# Autodesk Inventor assembly: s-assy-shooter_unit
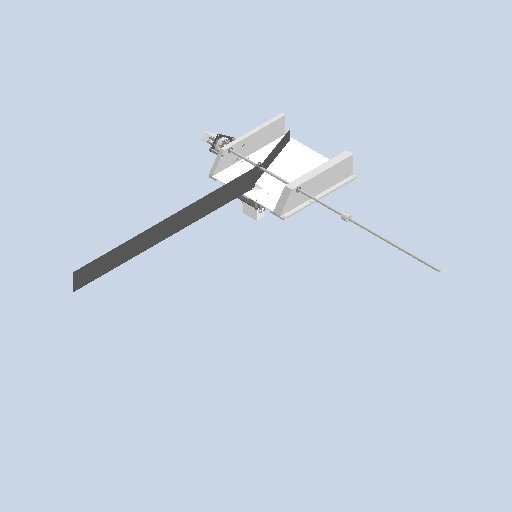
[picture p0: Inventor's stored thumbnail of the model, 512x512]
Saved by Autodesk Inventor 2022 (Build 260153000, 153)
## iProperties
Created: 2021-08-20
Part Number: s-assy-shooter_unit
Document SubType Name: Assembly
Designer: yuta0
Author: yuta0
## Documents named in this file (13)
- C:\Users\yuto6\Box\Public_Share\キャチロボバトルコンテスト2021\CAD\catchrobo_hardware\assy-shooter\s-assy-shooter_unit.iam
- C:\Users\yuto6\Box\Public_Share\キャチロボバトルコンテスト2021\CAD\catchrobo_hardware\assy-shooter\s_carbon_plate1.ipt
- C:\Users\yuto6\Box\Public_Share\キャチロボバトルコンテスト2021\CAD\catchrobo_hardware\assy-shooter\s_base2.ipt
- C:\Users\yuto6\Box\Public_Share\キャチロボバトルコンテスト2021\CAD\catchrobo_hardware\assy-shooter\s_base4.ipt
- C:\Users\yuto6\Box\Public_Share\キャチロボバトルコンテスト2021\CAD\catchrobo_hardware\assy-shooter\s-assy-guide_actuator.iam
- C:\Users\yuto6\Box\Public_Share\キャチロボバトルコンテスト2021\CAD\catchrobo_hardware\assy-shooter\MF126ZZ.ipt
- C:\Users\yuto6\Box\Public_Share\キャチロボバトルコンテスト2021\CAD\catchrobo_hardware\assy-shooter\CPRC16-6-6.iam
- C:\Users\yuto6\Box\Public_Share\キャチロボバトルコンテスト2021\CAD\catchrobo_hardware\assy-shooter\SCSTR6-8.iam
- C:\Users\yuto6\Box\Public_Share\キャチロボバトルコンテスト2021\CAD\catchrobo_hardware\assy-robot\CB4-10.ipt
- C:\Users\yuto6\Box\Public_Share\キャチロボバトルコンテスト2021\CAD\catchrobo_hardware\assy-shooter\s_carbon_plate5.ipt
- C:\Users\yuto6\Box\Public_Share\キャチロボバトルコンテスト2021\CAD\catchrobo_hardware\assy-shooter\s-assy-sorter.iam
- C:\Users\yuto6\Box\Public_Share\キャチロボバトルコンテスト2021\CAD\catchrobo_hardware\assy-shooter\PSFG6-350.ipt
- C:\Users\yuto6\Box\Public_Share\キャチロボバトルコンテスト2021\CAD\catchrobo_hardware\assy-shooter\PSFG6-270.ipt
## Components (17 placed, 12 different names)
1. s_base4:1 — メイト:20, メイト:21, フラッシュ:6, メイト:51, メイト:53, メイト:54, メイト:55, メイト:56, メイト:69, メイト:70, メイト:71, メイト:72, メイト:73, メイト:74, メイト:75, メイト:76, メイト:79
2. s-assy-guide_actuator:1 [sub-assembly] — メイト:51, メイト:69, メイト:70, フラッシュ:7
3. MF126ZZ:1 — メイト:53, メイト:54
4. MF126ZZ:2 — メイト:55, メイト:56
5. MF126ZZ:3 — メイト:58, メイト:59, メイト:83
6. MF126ZZ:4 — メイト:60, メイト:61, メイト:84
7. CPRC16-6-6:1 [sub-assembly] — メイト:65, メイト:84
8. CB4-10:1 — メイト:71, メイト:72
9. CB4-10:2 — メイト:73, メイト:74
10. CB4-10:3 — メイト:75, メイト:76
11. s_carbon_plate5:1 — メイト:78, メイト:79, 角度:1
12. SCSTR6-8:1 [sub-assembly] — メイト:78
13. s_base2:1 — メイト:13, メイト:14, フラッシュ:5, メイト:58, メイト:59, メイト:60, メイト:61, メイト:65
14. s_carbon_plate1:1 — メイト:13, メイト:14, メイト:20, メイト:21, フラッシュ:5, フラッシュ:6, メイト:80, メイト:81, メイト:82, 角度:1
15. s-assy-sorter:1 [sub-assembly] — メイト:80, メイト:81, メイト:82
16. PSFG6-350:1 — メイト:83, フラッシュ:7, メイト:85, メイト:86
17. PSFG6-270:1 — メイト:85, メイト:86
## Relationships (35: Mate 31, Flush 3, Angle 1)
- メイト:13 [Mate]: s_base2:1 ↔ s_carbon_plate1:1
- メイト:14 [Mate]: s_base2:1 ↔ s_carbon_plate1:1
- メイト:20 [Mate]: s_base4:1 ↔ s_carbon_plate1:1
- メイト:21 [Mate]: s_base4:1 ↔ s_carbon_plate1:1
- フラッシュ:5 [Flush]: s_base2:1 ↔ s_carbon_plate1:1
- フラッシュ:6 [Flush]: s_base4:1 ↔ s_carbon_plate1:1
- メイト:51 [Mate]: s_base4:1 ↔ s-assy-guide_actuator:1
- メイト:53 [Mate]: s_base4:1 ↔ MF126ZZ:1
- メイト:54 [Mate]: s_base4:1 ↔ MF126ZZ:1
- メイト:55 [Mate]: s_base4:1 ↔ MF126ZZ:2
- メイト:56 [Mate]: s_base4:1 ↔ MF126ZZ:2
- メイト:58 [Mate]: MF126ZZ:3 ↔ s_base2:1
- メイト:59 [Mate]: MF126ZZ:3 ↔ s_base2:1
- メイト:60 [Mate]: MF126ZZ:4 ↔ s_base2:1
- メイト:61 [Mate]: MF126ZZ:4 ↔ s_base2:1
- メイト:65 [Mate] (129.5 mm): CPRC16-6-6:1 ↔ s_base2:1
- メイト:69 [Mate]: s_base4:1 ↔ s-assy-guide_actuator:1
- メイト:70 [Mate]: s_base4:1 ↔ s-assy-guide_actuator:1
- メイト:71 [Mate]: s_base4:1 ↔ CB4-10:1
- メイト:72 [Mate]: s_base4:1 ↔ CB4-10:1
- メイト:73 [Mate]: s_base4:1 ↔ CB4-10:2
- メイト:74 [Mate]: s_base4:1 ↔ CB4-10:2
- メイト:75 [Mate]: s_base4:1 ↔ CB4-10:3
- メイト:76 [Mate]: s_base4:1 ↔ CB4-10:3
- メイト:78 [Mate]: s_carbon_plate5:1 ↔ SCSTR6-8:1
- メイト:79 [Mate] (87.5 mm): s_base4:1 ↔ s_carbon_plate5:1
- メイト:80 [Mate]: s_carbon_plate1:1 ↔ s-assy-sorter:1
- メイト:81 [Mate]: s_carbon_plate1:1 ↔ s-assy-sorter:1
- メイト:82 [Mate]: s_carbon_plate1:1 ↔ s-assy-sorter:1
- 角度:1 [Angle] (0 deg): s_carbon_plate5:1 ↔ s_carbon_plate1:1
- メイト:83 [Mate]: MF126ZZ:3 ↔ PSFG6-350:1
- フラッシュ:7 [Flush]: s-assy-guide_actuator:1 ↔ PSFG6-350:1
- メイト:84 [Mate]: MF126ZZ:4 ↔ CPRC16-6-6:1
- メイト:85 [Mate]: PSFG6-350:1 ↔ PSFG6-270:1
- メイト:86 [Mate]: PSFG6-350:1 ↔ PSFG6-270:1
